# Autodesk Inventor assembly: Assembly_KinematicMirror
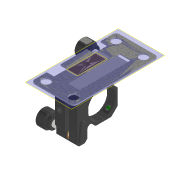
[picture p0: Inventor's stored thumbnail of the model, 180x180]
Saved by Autodesk Inventor 2022 (Build 260153000, 153)
## iProperties
Created: 2022-07-19
Part Number: Assembly_KinematicMirror
Document SubType Name: Assembly
Designer: wanghaoran
Author: wanghaoran
## Documents named in this file (3)
- E:\GitHub\SIMMO\INVENTOR\Assembly_KinematicMirror.iam
- E:\GitHub\SIMMO\INVENTOR\10_Mountinplate_Mirrors_v0.ipt
- E:\GitHub\SIMMO\INVENTOR\00_KM100-Step.ipt
## Components (2 placed, 2 different names)
1. 10_Mountinplate_Mirrors_v0:1 — Insert:1, Angle:1, Flush:1
2. 00_KM100-Step:1 — Insert:1, Angle:1
## Relationships (3: Insert 1, Angle 1, Flush 1)
- Insert:1: 10_Mountinplate_Mirrors_v0:1 ↔ 00_KM100-Step:1
- Angle:1 (0 deg): 10_Mountinplate_Mirrors_v0:1 ↔ 00_KM100-Step:1
- Flush:1 (-1.27 mm): 10_Mountinplate_Mirrors_v0:1
